# Autodesk Inventor assembly: LED Indicator Assem Farnell 1368996
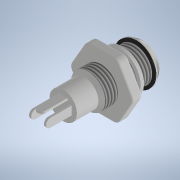
[picture p0: Inventor's stored thumbnail of the model, 180x180]
Saved by Autodesk Inventor 2021 (Build 250183000, 183)
## iProperties
Created: 2020-07-20
Part Number: LED Indicator Assem Farnell 1368996
Document SubType Name: Assembly
Designer: jgray
Author: jgray
## Documents named in this file (5)
- M:\Printed Electronics\Gas Sensors\Prototypes\Prototype II -Cartridge Reader V3\LED Indicator Assem Farnell 1368996.iam
- M:\Printed Electronics\Gas Sensors\Prototypes\Prototype II -Cartridge Reader V3\LED Indicator Farnell 19100054.ipt
- M:\Printed Electronics\Gas Sensors\Prototypes\Prototype II -Cartridge Reader V3\LED metal washer.ipt
- M:\Printed Electronics\Gas Sensors\Prototypes\Prototype II -Cartridge Reader V3\LED Nut.ipt
- M:\Printed Electronics\Gas Sensors\Prototypes\Prototype II -Cartridge Reader V3\LED washer.ipt
## Components (4 placed, 4 different names)
1. LED Indicator Farnell 19100054:1 — Mate:1, Mate:2, Mate:3, Mate:4
2. LED metal washer:1 — Mate:3
3. LED Nut:1 — Mate:4
4. LED washer:1 — Mate:1, Mate:2
## Relationships (4: Mate 4)
- Mate:1: LED Indicator Farnell 19100054:1 ↔ LED washer:1
- Mate:2: LED Indicator Farnell 19100054:1 ↔ LED washer:1
- Mate:3: LED Indicator Farnell 19100054:1 ↔ LED metal washer:1
- Mate:4: LED Indicator Farnell 19100054:1 ↔ LED Nut:1
